# Autodesk Inventor assembly: CY8CKIT-059
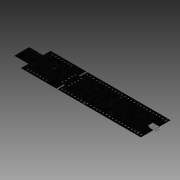
[picture p0: Inventor's stored thumbnail of the model, 180x180]
Saved by Autodesk Inventor 2018 (Build 220112000, 112)
## iProperties
Category: Loose
Company: Autodesk Inc.
Created: 2017-12-11
Part Number: CY8CKIT-059
Document SubType Name: Assembly
Designer: Autodesk Inc.
Catalog Web Link: http://www.cypress.com/documentation/development-kitsboards/cy8ckit-059-psoc-5lp-prototyping-kit
Vendor: Cypress
Author: Autodesk Inc.
Keywords: Gray tote
## Documents named in this file (3)
- D:\FIRST 2018\FIRST 2018 Inventor\FIRST 2018 Gray Tote\CY8CKIT-059.iam
- D:\FIRST 2018\FIRST 2018 Inventor\FIRST 2018 Gray Tote\Parts\fr16-030_ProtoKit.ipt
- D:\FIRST 2018\FIRST 2018 Inventor\FIRST 2018 Gray Tote\Parts\fc16-030_USB_PCB.ipt
## Components (2 placed, 2 different names)
1. fr16-030_ProtoKit:1 — Mate:1, Flush:1, Mate:3, Angle:2
2. fc16-030_USB_PCB:1 — Mate:1, Flush:1, Mate:2, Angle:1
## Relationships (7: Mate 4, Angle 2, Flush 1)
- Mate:1: fr16-030_ProtoKit:1 ↔ fc16-030_USB_PCB:1
- Flush:1 (-2 mm): fr16-030_ProtoKit:1 ↔ fc16-030_USB_PCB:1
- Mate:2: fc16-030_USB_PCB:1
- Angle:1 (0 deg): fc16-030_USB_PCB:1
- Mate:3: fr16-030_ProtoKit:1
- Angle:2 (0 deg): fr16-030_ProtoKit:1
- Mate:4
